# Autodesk Inventor assembly: センサ1セット
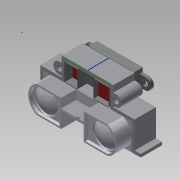
[picture p0: Inventor's stored thumbnail of the model, 180x180]
Saved by Autodesk Inventor 2017 (Build 210142000, 142)
## iProperties
Part Number: センサ1セット
Material: 一般
Document SubType Name: Assembly
Designer: HISAAKI
Author: HISAAKI
## Documents named in this file (4)
- C:\Users\HISAAKI\Documents\LYNCS\CanSat\2017種子島\cansat-structure\センサ1セット.iam
- C:\Users\HISAAKI\Documents\LYNCS\CanSat\2017種子島\cansat-structure\Sharp_2Y0A710.ipt
- C:\Users\HISAAKI\Documents\LYNCS\CanSat\2017種子島\cansat-structure\SharpDistanceRanger.ipt
- C:\Users\HISAAKI\Documents\LYNCS\CanSat\2017種子島\cansat-structure\センサ冶具1セット.ipt
## Components (3 placed, 3 different names)
1. SharpDistanceRanger:1 — メイト:3, メイト:5
2. センサ冶具1セット:1 — メイト:3, メイト:5, メイト:6, メイト:7, フラッシュ:1
3. Sharp_2Y0A710:1 — メイト:6, メイト:7, フラッシュ:1
## Relationships (5: Mate 4, Flush 1)
- メイト:3 [Mate]: SharpDistanceRanger:1 ↔ センサ冶具1セット:1
- メイト:5 [Mate]: SharpDistanceRanger:1 ↔ センサ冶具1セット:1
- メイト:6 [Mate]: センサ冶具1セット:1 ↔ Sharp_2Y0A710:1
- メイト:7 [Mate]: センサ冶具1セット:1 ↔ Sharp_2Y0A710:1
- フラッシュ:1 [Flush]: センサ冶具1セット:1 ↔ Sharp_2Y0A710:1
